# Autodesk Inventor assembly: Robomuse
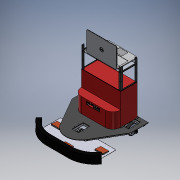
[picture p0: Inventor's stored thumbnail of the model, 180x180]
Saved by Autodesk Inventor 2018 (Build 220112000, 112)
## iProperties
Created: 2017-05-02
Part Number: Robomuse
Document SubType Name: Assembly
Designer: AYUSH SHUKLA
Author: AYUSH SHUKLA
## Documents named in this file (12)
- C:\Study\BTP2\Robomuse Inventor CAD\Robomuse.iam
- C:\Study\BTP2\Robomuse Inventor CAD\Chassis_2.ipt
- C:\Study\BTP2\Robomuse Inventor CAD\Acrylic_base_1.ipt
- C:\Study\BTP2\Robomuse Inventor CAD\shell.ipt
- C:\Study\BTP2\Robomuse Inventor CAD\kinect\Kinect.iam
- C:\Study\BTP2\Robomuse Inventor CAD\rack\rack.iam
- C:\Study\BTP2\Robomuse Inventor CAD\castor\castor.iam
- C:\Study\BTP2\Robomuse Inventor CAD\motor_wheel\motor_wheel.iam
- C:\Study\BTP2\Robomuse Inventor CAD\Battery.ipt
- C:\Study\BTP2\Robomuse Inventor CAD\encoder\amt112q-v.iam
- C:\Study\BTP2\Robomuse Inventor CAD\Laptop.ipt
- C:\Study\BTP2\Robomuse Inventor CAD\Charging Dock.ipt
## Components (14 placed, 11 different names)
1. Chassis_2:1 — Mate:3, Mate:117, Mate:118, Mate:119, Mate:120, Mate:121, Mate:123, Mate:124, Mate:125, Mate:126, Mate:136, Mate:137, Flush:10
2. Acrylic_base_1:1 — Mate:3, Mate:93, Mate:114, Mate:127, Mate:128, Mate:136, Mate:137, Mate:138, Angle:3, Flush:11
3. shell:1 — Mate:93, Mate:111, Mate:112, Mate:113, Mate:115, Mate:116
4. Kinect:1 [sub-assembly] — Mate:111, Mate:112, Mate:113
5. rack:1 [sub-assembly] — Mate:114, Mate:115, Mate:116, Mate:129, Mate:130, Flush:5, Flush:6, Mate:135, Flush:7, Flush:8, Mate:138, Flush:11
6. castor:1 [sub-assembly] — Mate:117, Mate:118, Mate:119
7. motor_wheel:1 [sub-assembly] — Mate:120, Mate:121, Mate:125, Mate:133, Mate:134, Angle:1, Tangent:1
8. motor_wheel:2 [sub-assembly] — Mate:123, Mate:124, Mate:126, Mate:131, Mate:132, Angle:2
9. Battery:1 — Mate:127, Mate:129, Flush:6
10. Battery:2 — Mate:128, Mate:130, Flush:5
11. amt112q-v:1 [sub-assembly] — Mate:131, Mate:132, Angle:2
12. amt112q-v:2 [sub-assembly] — Mate:133, Mate:134, Angle:1
13. Laptop:1 — Mate:135, Flush:7, Flush:8
14. Charging Dock:1 — Mate:139, Angle:4, Flush:12
## Relationships (42: Mate 30, Flush 7, Angle 4, Tangent 1)
- Mate:3: Chassis_2:1 ↔ Acrylic_base_1:1
- Mate:93: Acrylic_base_1:1 ↔ shell:1
- Mate:111: shell:1 ↔ Kinect:1
- Mate:112 (10 mm): shell:1 ↔ Kinect:1
- Mate:113 (85 mm): shell:1 ↔ Kinect:1
- Mate:114: Acrylic_base_1:1 ↔ rack:1
- Mate:115: shell:1 ↔ rack:1
- Mate:116: shell:1 ↔ rack:1
- Mate:117: Chassis_2:1 ↔ castor:1
- Mate:118: Chassis_2:1 ↔ castor:1
- Mate:119: Chassis_2:1 ↔ castor:1
- Mate:120: Chassis_2:1 ↔ motor_wheel:1
- Mate:121: Chassis_2:1 ↔ motor_wheel:1
- Mate:123: Chassis_2:1 ↔ motor_wheel:2
- Mate:124: Chassis_2:1 ↔ motor_wheel:2
- Mate:125: Chassis_2:1 ↔ motor_wheel:1
- Mate:126: Chassis_2:1 ↔ motor_wheel:2
- Mate:127: Acrylic_base_1:1 ↔ Battery:1
- Mate:128: Acrylic_base_1:1 ↔ Battery:2
- Mate:129: rack:1 ↔ Battery:1
- Mate:130: rack:1 ↔ Battery:2
- Flush:5: rack:1 ↔ Battery:2
- Flush:6: rack:1 ↔ Battery:1
- Mate:131: motor_wheel:2 ↔ amt112q-v:1
- Mate:132: motor_wheel:2 ↔ amt112q-v:1
- Mate:133: motor_wheel:1 ↔ amt112q-v:2
- Mate:134: motor_wheel:1 ↔ amt112q-v:2
- Angle:1 (0 deg): motor_wheel:1 ↔ amt112q-v:2
- Angle:2 (180 deg): motor_wheel:2 ↔ amt112q-v:1
- Mate:135: rack:1 ↔ Laptop:1
- Flush:7 (53 mm): rack:1 ↔ Laptop:1
- Flush:8: rack:1 ↔ Laptop:1
- Mate:136: Chassis_2:1 ↔ Acrylic_base_1:1
- Mate:137: Chassis_2:1 ↔ Acrylic_base_1:1
- Mate:138 (-37.7455 mm): Acrylic_base_1:1 ↔ rack:1
- Angle:3 (0 deg): Acrylic_base_1:1
- Tangent:1: motor_wheel:1
- Mate:139: Charging Dock:1
- Angle:4 (0 deg): Charging Dock:1
- Flush:10 (-350 mm): Chassis_2:1
- Flush:11 (-5 mm): Acrylic_base_1:1 ↔ rack:1
- Flush:12 (-350 mm): Charging Dock:1
